# Autodesk Inventor assembly: stepperMotorAndYokeEndTemp
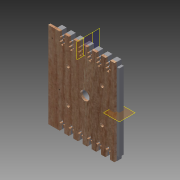
[picture p0: Inventor's stored thumbnail of the model, 180x180]
Saved by Autodesk Inventor 2013 (Build 170138000, 138)
## iProperties
Created: 2013-02-24
Part Number: stepperMotorAndYokeEndTemp
Document SubType Name: Assembly
Designer: Nano
Author: Nano
## Documents named in this file (3)
- C:\Users\Nano\Documents\InventorByron\InventorMasterProject\gyroPhone01\stepperMotorAndYokeEndTemp.iam
- C:\Users\Nano\Documents\InventorByron\InventorMasterProject\gyroPhone01\yokeEndBlock.ipt
- C:\Users\Nano\Documents\InventorByron\InventorMasterProject\gyroPhone01\gearAssemblyTake02\stepperMotorMountPlate01.ipt
## Components (2 placed, 2 different names)
1. yokeEndBlock:1 — Mate:1, Flush:1, Mate:2
2. stepperMotorMountPlate01:1 — Mate:1, Flush:1, Mate:2
## Relationships (3: Mate 2, Flush 1)
- Mate:1: yokeEndBlock:1 ↔ stepperMotorMountPlate01:1
- Flush:1: yokeEndBlock:1 ↔ stepperMotorMountPlate01:1
- Mate:2: yokeEndBlock:1 ↔ stepperMotorMountPlate01:1
